# Autodesk Inventor assembly: F606ZZ
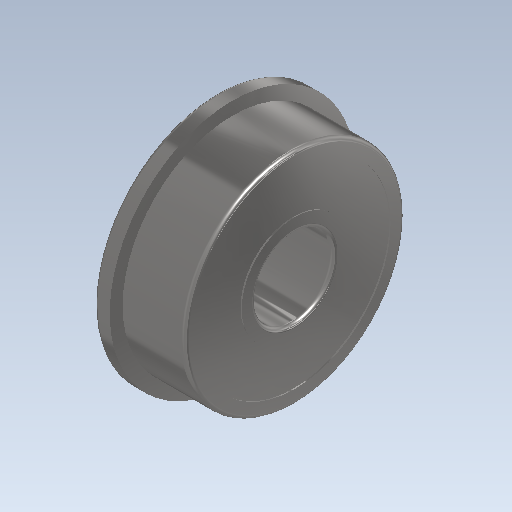
[picture p0: Inventor's stored thumbnail of the model, 512x512]
Saved by Autodesk Inventor 2020.3 (Build 243373000, 373)
## iProperties
Part Number: F606ZZ
Catalog Web Link: www.cadenas.de
Description: Shielded Type ZZ-ZZS-
Vendor: NSK_RB
Document SubType Name: Assembly
Designer: partserver
Manufacturer: NSK_RB
Mass: 6.91669 g
Surface Area: 19.9933 cm^2
Volume: 0.881107 cm^3
Density: 7.85 g/cm^3
Category: PARTsolutions
Company: NSK_RB
PSOL_IDENT_0: {$CADENAS_DATA\23d-libs\nsk_rb\roller_bearings\deep_groove_bb\exstra_small_miniatur_bb\metric_design
PSOL_IDENT_1: _with_flange\shielded_type_zz_zzs_1_asmtab.prj},172 {VTYP=3D},{STYP=ASSTAB},{NB=F606ZZ},{LINA=F606ZZ
PSOL_IDENT_2: },{NN=Shielded Type ZZ-ZZS},{DATE=10.04.2020 04:57:39},{GEOMDATE=04.01.2008},{VERSION=},{LINEID=540}
PSOL_IDENT_3: ,{WBVAR=},{WBNUMERIC=}  {NB=F606ZZ},{LINA=F606ZZ},{KT=DUMMY},{IDNR=},{STAN=-},{ORDER=F606ZZ},{SD=6.0
PSOL_IDENT_4: },{X=6.0},{D=17},{DD=17},{DD1=0.0},{D2=19.0},{DD2=19.0},{B=0.0},{B1=6.0},{CC1=0.0},{C2=1.2},{CC2=1.2
PSOL_IDENT_5: },{R=0.00},{R1=0.30},{DI1=8.92},{DI2=8.20},{SDE1=13.75},{SDE2=14.80},{CR1=2260},{COR1=835},{CR2=231}
PSOL_IDENT_6: ,{COR2=85.0},{LG=38000},{LO=45000},{DA=0.0},{DB=8.2},{RA=0.00},{RB=0.30},{MASS=6.61},{SC=1},{PPATH=s
PSOL_IDENT_7: hielded_type_zz_zzs_asmtpl.prj}
NB: F606ZZ
NN: Shielded Type ZZ-ZZS
NBSYN: $ORDER.
LINA: F606ZZ
CATALOG: NSK Rolling Bearing
STAN: -
ORDER: F606ZZ
SD: 6
D: 17
D2: 19
B1: 6
C2: 1.2
R1: 0.3
CR1: 2260
COR1: 835
CR2: 231
COR2: 85
LG: 38000
DB: 8.2
RB: 0.3
MASS: 6.61
SUPPLIER: NSK_RB
ARTICLENO: F606ZZ
BOMINFO: F606ZZ
CREATOR: CADENAS GmbH
Title: F606ZZ
Author: Cadenas PARTsolutions
## Documents named in this file (6)
- D:\mysvn\ロボコン\キャチロボ\キャチロボ設計図\ロボット\共有パーツ\F606ZZ\F606ZZ.iam
- D:\mysvn\ロボコン\キャチロボ\キャチロボ設計図\ロボット\共有パーツ\F606ZZ\F606ZZ Outer Ring.ipt
- D:\mysvn\ロボコン\キャチロボ\キャチロボ設計図\ロボット\共有パーツ\F606ZZ\F606ZZ Inner Ring.ipt
- D:\mysvn\ロボコン\キャチロボ\キャチロボ設計図\ロボット\共有パーツ\F606ZZ\F606ZZ Shield1.ipt
- D:\mysvn\ロボコン\キャチロボ\キャチロボ設計図\ロボット\共有パーツ\F606ZZ\F606ZZ Ball.ipt
- D:\mysvn\ロボコン\キャチロボ\キャチロボ設計図\ロボット\共有パーツ\F606ZZ\F606ZZ Shield2.ipt
## Components (12 placed, 5 different names)
1. F606ZZ Outer Ring:1 — ip_st_1_XY@1 <-> ip_st_1a_XY@2, ip_st_1_Z@1 <-> ip_st_1a_Z@2, ip_st_1_YZ@1 <-> ip_st_1a_YZ@2, ip_st_2_XY@1 <-> ip_st_1_XY@12, ip_st_2_Z@1 <-> ip_st_1_Z@12, ip_st_2_YZ@1 <-> ip_st_1_YZ@12
2. F606ZZ Inner Ring:1 — ip_st_1_XY@1 <-> ip_st_1a_XY@2, ip_st_1_Z@1 <-> ip_st_1a_Z@2, ip_st_1_YZ@1 <-> ip_st_1a_YZ@2, ip_st_2a_XY@2 <-> ip_st_1_XY@3, ip_st_2a_Z@2 <-> ip_st_1_Z@3, ip_st_2a_YZ@2 <-> ip_st_1_YZ@3, ip_st_1_1_XY@2 <-> ip_st_1_XY@4, ip_st_1_1_Z@2 <-> ip_st_1_Z@4, ip_st_1_1_YZ@2 <-> ip_st_1_YZ@4, ip_st_1_2_XY@2 <-> ip_st_1_XY@5, ip_st_1_2_Z@2 <-> ip_st_1_Z@5, ip_st_1_2_YZ@2 <-> ip_st_1_YZ@5, ip_st_1_3_XY@2 <-> ip_st_1_XY@6, ip_st_1_3_Z@2 <-> ip_st_1_Z@6, ip_st_1_3_YZ@2 <-> ip_st_1_YZ@6, ip_st_1_4_XY@2 <-> ip_st_1_XY@7, ip_st_1_4_Z@2 <-> ip_st_1_Z@7, ip_st_1_4_YZ@2 <-> ip_st_1_YZ@7, ip_st_1_5_XY@2 <-> ip_st_1_XY@8, ip_st_1_5_Z@2 <-> ip_st_1_Z@8, ip_st_1_5_YZ@2 <-> ip_st_1_YZ@8, ip_st_1_6_XY@2 <-> ip_st_1_XY@9, ip_st_1_6_Z@2 <-> ip_st_1_Z@9, ip_st_1_6_YZ@2 <-> ip_st_1_YZ@9, ip_st_1_7_XY@2 <-> ip_st_1_XY@10, ip_st_1_7_Z@2 <-> ip_st_1_Z@10, ip_st_1_7_YZ@2 <-> ip_st_1_YZ@10, ip_st_1_8_XY@2 <-> ip_st_1_XY@11, ip_st_1_8_Z@2 <-> ip_st_1_Z@11, ip_st_1_8_YZ@2 <-> ip_st_1_YZ@11
3. F606ZZ Shield1:1 — ip_st_2a_XY@2 <-> ip_st_1_XY@3, ip_st_2a_Z@2 <-> ip_st_1_Z@3, ip_st_2a_YZ@2 <-> ip_st_1_YZ@3
4. F606ZZ Ball:1 — ip_st_1_1_XY@2 <-> ip_st_1_XY@4, ip_st_1_1_Z@2 <-> ip_st_1_Z@4, ip_st_1_1_YZ@2 <-> ip_st_1_YZ@4
5. F606ZZ Ball:2 — ip_st_1_2_XY@2 <-> ip_st_1_XY@5, ip_st_1_2_Z@2 <-> ip_st_1_Z@5, ip_st_1_2_YZ@2 <-> ip_st_1_YZ@5
6. F606ZZ Ball:3 — ip_st_1_3_XY@2 <-> ip_st_1_XY@6, ip_st_1_3_Z@2 <-> ip_st_1_Z@6, ip_st_1_3_YZ@2 <-> ip_st_1_YZ@6
7. F606ZZ Ball:4 — ip_st_1_4_XY@2 <-> ip_st_1_XY@7, ip_st_1_4_Z@2 <-> ip_st_1_Z@7, ip_st_1_4_YZ@2 <-> ip_st_1_YZ@7
8. F606ZZ Ball:5 — ip_st_1_5_XY@2 <-> ip_st_1_XY@8, ip_st_1_5_Z@2 <-> ip_st_1_Z@8, ip_st_1_5_YZ@2 <-> ip_st_1_YZ@8
9. F606ZZ Ball:6 — ip_st_1_6_XY@2 <-> ip_st_1_XY@9, ip_st_1_6_Z@2 <-> ip_st_1_Z@9, ip_st_1_6_YZ@2 <-> ip_st_1_YZ@9
10. F606ZZ Ball:7 — ip_st_1_7_XY@2 <-> ip_st_1_XY@10, ip_st_1_7_Z@2 <-> ip_st_1_Z@10, ip_st_1_7_YZ@2 <-> ip_st_1_YZ@10
11. F606ZZ Ball:8 — ip_st_1_8_XY@2 <-> ip_st_1_XY@11, ip_st_1_8_Z@2 <-> ip_st_1_Z@11, ip_st_1_8_YZ@2 <-> ip_st_1_YZ@11
12. F606ZZ Shield2:1 — ip_st_2_XY@1 <-> ip_st_1_XY@12, ip_st_2_Z@1 <-> ip_st_1_Z@12, ip_st_2_YZ@1 <-> ip_st_1_YZ@12
## Relationships (33: Mate 20, Angle 11, Flush 2)
- ip_st_1_XY@1 <-> ip_st_1a_XY@2 [Flush]: F606ZZ Outer Ring:1 ↔ F606ZZ Inner Ring:1
- ip_st_1_Z@1 <-> ip_st_1a_Z@2 [Mate]: F606ZZ Outer Ring:1 ↔ F606ZZ Inner Ring:1
- ip_st_1_YZ@1 <-> ip_st_1a_YZ@2 [Angle] (90 deg): F606ZZ Outer Ring:1 ↔ F606ZZ Inner Ring:1
- ip_st_2a_XY@2 <-> ip_st_1_XY@3 [Flush]: F606ZZ Inner Ring:1 ↔ F606ZZ Shield1:1
- ip_st_2a_Z@2 <-> ip_st_1_Z@3 [Mate]: F606ZZ Inner Ring:1 ↔ F606ZZ Shield1:1
- ip_st_2a_YZ@2 <-> ip_st_1_YZ@3 [Angle] (0 deg): F606ZZ Inner Ring:1 ↔ F606ZZ Shield1:1
- ip_st_1_1_XY@2 <-> ip_st_1_XY@4 [Mate]: F606ZZ Inner Ring:1 ↔ F606ZZ Ball:1
- ip_st_1_1_Z@2 <-> ip_st_1_Z@4 [Mate]: F606ZZ Inner Ring:1 ↔ F606ZZ Ball:1
- ip_st_1_1_YZ@2 <-> ip_st_1_YZ@4 [Angle] (0 deg): F606ZZ Inner Ring:1 ↔ F606ZZ Ball:1
- ip_st_1_2_XY@2 <-> ip_st_1_XY@5 [Mate]: F606ZZ Inner Ring:1 ↔ F606ZZ Ball:2
- ip_st_1_2_Z@2 <-> ip_st_1_Z@5 [Mate]: F606ZZ Inner Ring:1 ↔ F606ZZ Ball:2
- ip_st_1_2_YZ@2 <-> ip_st_1_YZ@5 [Angle] (0 deg): F606ZZ Inner Ring:1 ↔ F606ZZ Ball:2
- ip_st_1_3_XY@2 <-> ip_st_1_XY@6 [Mate]: F606ZZ Inner Ring:1 ↔ F606ZZ Ball:3
- ip_st_1_3_Z@2 <-> ip_st_1_Z@6 [Mate]: F606ZZ Inner Ring:1 ↔ F606ZZ Ball:3
- ip_st_1_3_YZ@2 <-> ip_st_1_YZ@6 [Angle] (0 deg): F606ZZ Inner Ring:1 ↔ F606ZZ Ball:3
- ip_st_1_4_XY@2 <-> ip_st_1_XY@7 [Mate]: F606ZZ Inner Ring:1 ↔ F606ZZ Ball:4
- ip_st_1_4_Z@2 <-> ip_st_1_Z@7 [Mate]: F606ZZ Inner Ring:1 ↔ F606ZZ Ball:4
- ip_st_1_4_YZ@2 <-> ip_st_1_YZ@7 [Angle] (0 deg): F606ZZ Inner Ring:1 ↔ F606ZZ Ball:4
- ip_st_1_5_XY@2 <-> ip_st_1_XY@8 [Mate]: F606ZZ Inner Ring:1 ↔ F606ZZ Ball:5
- ip_st_1_5_Z@2 <-> ip_st_1_Z@8 [Mate]: F606ZZ Inner Ring:1 ↔ F606ZZ Ball:5
- ip_st_1_5_YZ@2 <-> ip_st_1_YZ@8 [Angle] (0 deg): F606ZZ Inner Ring:1 ↔ F606ZZ Ball:5
- ip_st_1_6_XY@2 <-> ip_st_1_XY@9 [Mate]: F606ZZ Inner Ring:1 ↔ F606ZZ Ball:6
- ip_st_1_6_Z@2 <-> ip_st_1_Z@9 [Mate]: F606ZZ Inner Ring:1 ↔ F606ZZ Ball:6
- ip_st_1_6_YZ@2 <-> ip_st_1_YZ@9 [Angle] (0 deg): F606ZZ Inner Ring:1 ↔ F606ZZ Ball:6
- ip_st_1_7_XY@2 <-> ip_st_1_XY@10 [Mate]: F606ZZ Inner Ring:1 ↔ F606ZZ Ball:7
- ip_st_1_7_Z@2 <-> ip_st_1_Z@10 [Mate]: F606ZZ Inner Ring:1 ↔ F606ZZ Ball:7
- ip_st_1_7_YZ@2 <-> ip_st_1_YZ@10 [Angle] (0 deg): F606ZZ Inner Ring:1 ↔ F606ZZ Ball:7
- ip_st_1_8_XY@2 <-> ip_st_1_XY@11 [Mate]: F606ZZ Inner Ring:1 ↔ F606ZZ Ball:8
- ip_st_1_8_Z@2 <-> ip_st_1_Z@11 [Mate]: F606ZZ Inner Ring:1 ↔ F606ZZ Ball:8
- ip_st_1_8_YZ@2 <-> ip_st_1_YZ@11 [Angle] (0 deg): F606ZZ Inner Ring:1 ↔ F606ZZ Ball:8
- ip_st_2_XY@1 <-> ip_st_1_XY@12 [Mate]: F606ZZ Outer Ring:1 ↔ F606ZZ Shield2:1
- ip_st_2_Z@1 <-> ip_st_1_Z@12 [Mate]: F606ZZ Outer Ring:1 ↔ F606ZZ Shield2:1
- ip_st_2_YZ@1 <-> ip_st_1_YZ@12 [Angle] (0 deg): F606ZZ Outer Ring:1 ↔ F606ZZ Shield2:1
